# Autodesk Inventor assembly: Assembly1
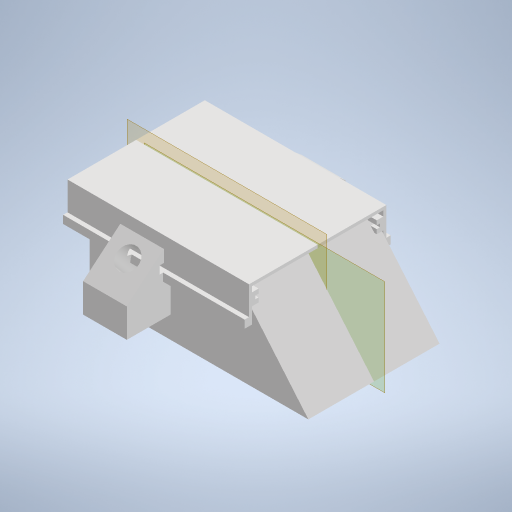
[picture p0: Inventor's stored thumbnail of the model, 512x512]
Saved by Autodesk Inventor 2023 (Build 270158000, 158)
## iProperties
Created: 2023-03-22
Part Number: Assembly1
Document SubType Name: Assembly
Designer: Umut Yücesoy
Author: Umut Yücesoy
## Documents named in this file (3)
- C:\Users\ycsyy\Desktop\kumanda kabza\Assembly1.iam
- C:\Users\ycsyy\Desktop\kumanda kabza\taslak2.ipt
- C:\Users\ycsyy\Desktop\kumanda kabza\kabza başlık.ipt
## Components (2 placed, 2 different names)
1. taslak2:1 — Mate:1
2. kabza başlık:1 — Mate:1
## Relationships (1: Mate 1)
- Mate:1: taslak2:1 ↔ kabza başlık:1
